# Autodesk Inventor assembly: #Turret
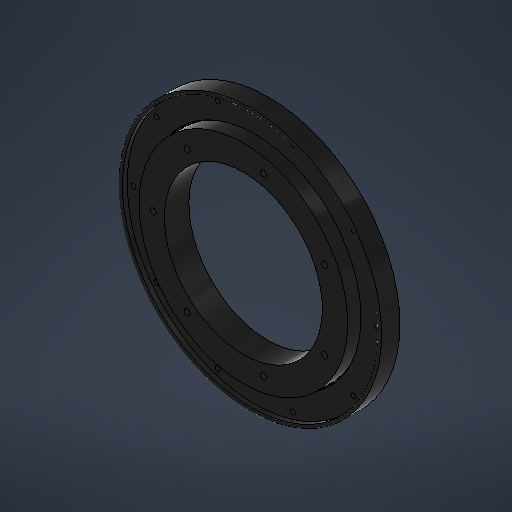
[picture p0: Inventor's stored thumbnail of the model, 512x512]
Saved by Autodesk Inventor 2026 (Build 300175000, 175)
## iProperties
Created: 2026-02-01
Part Number: #Turret
Document SubType Name: Assembly
Designer: Owen L
Mass: 661.765 g
Surface Area: 1768.58 cm^2
Volume: 441.737 cm^3
Density: 1.4981 g/cm^3
Author: Owen L
## Documents named in this file (3)
- C:\Users\littl\OneDrive\Documents\GitHub\2026-Robot-Mechanical\Shooter\Turret\#Turret.iam
- C:\Users\littl\OneDrive\Documents\GitHub\2026-Robot-Mechanical\Shooter\Turret\3DPRINT,TURRET,BEARING,INNER.ipt
- C:\Users\littl\OneDrive\Documents\GitHub\2026-Robot-Mechanical\Shooter\Turret\3DPRINT,TURRET,BEARING,OUTER.ipt
## Components (2 placed, 2 different names)
1. 3DPRINT,TURRET,BEARING,INNER:1 — Flush:1, Mate:1
2. 3DPRINT,TURRET,BEARING,OUTER:1 — Flush:1, Mate:1
## Relationships (2: Flush 1, Mate 1)
- Flush:1 (-0.7937 mm): 3DPRINT,TURRET,BEARING,INNER:1 ↔ 3DPRINT,TURRET,BEARING,OUTER:1
- Mate:1: 3DPRINT,TURRET,BEARING,INNER:1 ↔ 3DPRINT,TURRET,BEARING,OUTER:1
